# Autodesk Inventor assembly: ASM IMU
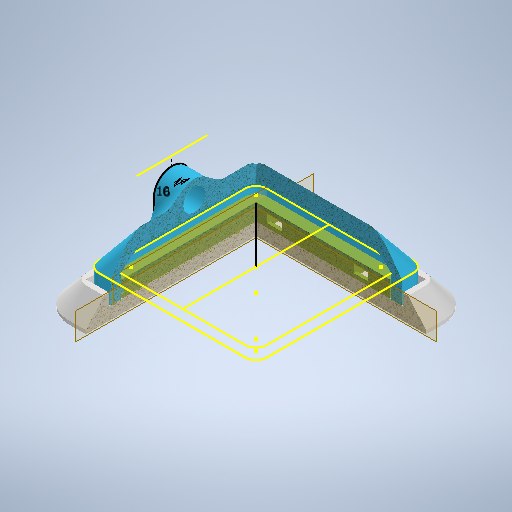
[picture p0: Inventor's stored thumbnail of the model, 512x512]
Saved by Autodesk Inventor 2025.2 (Build 292293000, 293)
## iProperties
Created: 2024-11-17
Part Number: ASM IMU
Document SubType Name: Assembly
Designer: tills
Author: tills
## Documents named in this file (4)
- C:\Users\tills\Desktop\Studium\Semester_3\Repositorys\Wearable-Health-Device\Inventor_AKTUELL\ASM IMU.iam
- C:\Users\tills\Desktop\Studium\Semester_3\Repositorys\Wearable-Health-Device\Inventor_AKTUELL\IMU_Base_T-Shirt.ipt
- C:\Users\tills\Desktop\Studium\Semester_3\Repositorys\Wearable-Health-Device\Inventor_AKTUELL\IMU_mount_baseplate.ipt
- C:\Users\tills\Desktop\Studium\Semester_3\Repositorys\Wearable-Health-Device\Inventor_AKTUELL\IMU_mount_cover.ipt
## Components (3 placed, 3 different names)
1. IMU_Base_T-Shirt:1 — Passend:1, Passend:2, Passend:3, Passend:4, Passend:5, Passend:6, Fluchtend:1, Fluchtend:2
2. IMU_mount_baseplate:1 — Passend:1, Passend:2, Passend:3
3. IMU_mount_cover:1 — Passend:4, Passend:5, Passend:6
## Relationships (8: Mate 6, Flush 2)
- Passend:1 [Mate] (3.5 mm): IMU_Base_T-Shirt:1 ↔ IMU_mount_baseplate:1
- Passend:2 [Mate] (3.5 mm): IMU_Base_T-Shirt:1 ↔ IMU_mount_baseplate:1
- Passend:3 [Mate]: IMU_Base_T-Shirt:1 ↔ IMU_mount_baseplate:1
- Passend:4 [Mate] (0.25 mm): IMU_Base_T-Shirt:1 ↔ IMU_mount_cover:1
- Passend:5 [Mate] (0.25 mm): IMU_Base_T-Shirt:1 ↔ IMU_mount_cover:1
- Passend:6 [Mate]: IMU_Base_T-Shirt:1 ↔ IMU_mount_cover:1
- Fluchtend:1 [Flush] (-17 mm): IMU_Base_T-Shirt:1
- Fluchtend:2 [Flush] (-17 mm): IMU_Base_T-Shirt:1
